# Autodesk Inventor assembly: Ensamble robot
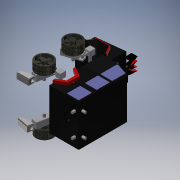
[picture p0: Inventor's stored thumbnail of the model, 180x180]
Saved by Autodesk Inventor 2017 (Build 210142000, 142)
## iProperties
Part Number: Ensamble robot
Material: Genérico
Document SubType Name: Assembly
Designer: HOME
Author: HOME
## Documents named in this file (9)
- C:\Users\HOME\Desktop\Transformer\Transformer\Ensamble robot.iam
- C:\Users\HOME\Desktop\Transformer\Transformer\Carro\Bumper.ipt
- C:\Users\HOME\Desktop\Transformer\Transformer\NuevoProyecto\PuertaMarco.iam
- C:\Users\HOME\Desktop\Transformer\Transformer\Hombro.ipt
- C:\Users\HOME\Desktop\Transformer\Transformer\Union pie.ipt
- C:\Users\HOME\Desktop\Transformer\Transformer\Ante pierna.ipt
- C:\Users\HOME\Desktop\Transformer\Transformer\Pie.ipt
- C:\Users\HOME\Downloads\llanta xddd.ipt
- C:\Users\HOME\Desktop\Transformer\Transformer\CabezaCarro.ipt
## Components (23 placed, 8 different names)
1. PuertaMarco:1 [sub-assembly] — Plana:1, Rígido:5, Rígido:6, Rígido:8
2. Bumper:1 — Plana:1, Rígido:1, Rígido:2, Rígido:8, Rígido:15
3. Union pie:1 — Rígido:3, De rotación:2
4. Hombro:3 — Rígido:1, Rígido:4
5. Hombro:4 — Rígido:2, Rígido:3
6. Union pie:2 — Rígido:4, De rotación:1
7. Ante pierna:1 — De rotación:1, Rígido:12
8. Ante pierna:2 — De rotación:2, De rotación:8
9. Hombro:5 — Rígido:6, Rígido:9
10. Hombro:6 — Rígido:5, Rígido:7
11. Union pie:3 — Rígido:7, De rotación:4
12. Ante pierna:3 — De rotación:4, Rígido:10, Rígido:13
13. Union pie:4 — Rígido:9, De rotación:5
14. Ante pierna:4 — De rotación:5, Rígido:11, Rígido:14
15. Union pie:5 — Rígido:11, De rotación:7
16. Union pie:6 — Rígido:10, De rotación:6
17. Pie:1 — De rotación:7
18. Pie:2 — De rotación:6
19. llanta xddd:1 — Rígido:13
20. llanta xddd:2 — Rígido:12
21. llanta xddd:3 — De rotación:8
22. llanta xddd:4 — Rígido:14
23. CabezaCarro:2 — Rígido:15
## Relationships (23: WeldJoint 15, RevoluteJoint 7, PlanarJoint 1)
- Plana:1: PuertaMarco:1 ↔ Bumper:1
- Rígido:1 [WeldJoint]: Bumper:1 ↔ Hombro:3
- Rígido:2 [WeldJoint]: Bumper:1 ↔ Hombro:4
- Rígido:3 [WeldJoint]: Union pie:1 ↔ Hombro:4
- Rígido:4 [WeldJoint]: Hombro:3 ↔ Union pie:2
- De rotación:1 [RevoluteJoint]: Union pie:2 ↔ Ante pierna:1
- De rotación:2 [RevoluteJoint]: Union pie:1 ↔ Ante pierna:2
- Rígido:5 [WeldJoint]: PuertaMarco:1 ↔ Hombro:6
- Rígido:6 [WeldJoint]: PuertaMarco:1 ↔ Hombro:5
- Rígido:7 [WeldJoint]: Hombro:6 ↔ Union pie:3
- De rotación:4 [RevoluteJoint]: Union pie:3 ↔ Ante pierna:3
- Rígido:8 [WeldJoint]: PuertaMarco:1 ↔ Bumper:1
- Rígido:9 [WeldJoint]: Hombro:5 ↔ Union pie:4
- De rotación:5 [RevoluteJoint]: Union pie:4 ↔ Ante pierna:4
- Rígido:10 [WeldJoint]: Ante pierna:3 ↔ Union pie:6
- Rígido:11 [WeldJoint]: Ante pierna:4 ↔ Union pie:5
- De rotación:6 [RevoluteJoint]: Union pie:6 ↔ Pie:2
- De rotación:7 [RevoluteJoint]: Union pie:5 ↔ Pie:1
- Rígido:12 [WeldJoint]: Ante pierna:1 ↔ llanta xddd:2
- De rotación:8 [RevoluteJoint]: Ante pierna:2 ↔ llanta xddd:3
- Rígido:13 [WeldJoint]: Ante pierna:3 ↔ llanta xddd:1
- Rígido:14 [WeldJoint]: Ante pierna:4 ↔ llanta xddd:4
- Rígido:15 [WeldJoint]: Bumper:1 ↔ CabezaCarro:2
